# Autodesk Inventor assembly: OpenROV_Dev_EChassis
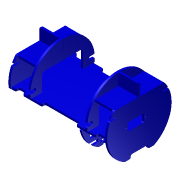
[picture p0: Inventor's stored thumbnail of the model, 180x180]
Saved by Autodesk Inventor 2012 (Build 160160000, 160)
## iProperties
Created: 2012-07-04
Part Number: OpenROV_Dev_EChassis
Document SubType Name: Assembly
Designer: user
Author: user
## Documents named in this file (9)
- C:\Users\user\Desktop\CLEAN ME\OpenROV\openrov-hardware\OpenROV 2.3.2 Dev\OpenROV_Dev_EChassis.iam
- C:\Users\user\Desktop\CLEAN ME\OpenROV\openrov-hardware\OpenROV 2.3.2 Dev\OpenROV_Dev_EChassis_Main_Plate.ipt
- C:\Users\user\Desktop\CLEAN ME\OpenROV\openrov-hardware\OpenROV 2.3.2 Dev\OpenROV_Dev_EChassis_Blinder.ipt
- C:\Users\user\Desktop\CLEAN ME\OpenROV\openrov-hardware\OpenROV 2.3.2 Dev\OpenROV_Dev_EChassis_Servo_Plate.ipt
- C:\Users\user\Desktop\CLEAN ME\OpenROV\openrov-hardware\OpenROV 2.3.2 Dev\OpenROV_Dev_EChassis_Plug_Mount.ipt
- C:\Users\user\Desktop\CLEAN ME\OpenROV\openrov-hardware\OpenROV 2.3.2 Dev\OpenROV_Dev_EChassis_Seperator.ipt
- C:\Users\user\Desktop\CLEAN ME\OpenROV\openrov-hardware\OpenROV 2.3.2 Dev\OpenROV_Dev_EChassis_Pivot_Plate.ipt
- C:\Users\user\Desktop\CLEAN ME\OpenROV\openrov-hardware\OpenROV 2.3.2 Dev\OpenROV_Dev_EChassis_Light_Plate.ipt
- C:\Users\user\Desktop\CLEAN ME\OpenROV\openrov-hardware\OpenROV 2.3.2 Dev\OpenROV_Dev_EChassis_Horz_Blinder.ipt
## Components (12 placed, 8 different names)
1. OpenROV_Dev_EChassis_Main_Plate:1 — Mate:1, Mate:2, Mate:3, Mate:4, Mate:5, Mate:6, Mate:7, Mate:8, Mate:9, Mate:10, Mate:11, Mate:12, Mate:13, Mate:14, Mate:15, Mate:16, Mate:19, Mate:20, Mate:21
2. OpenROV_Dev_EChassis_Blinder:1 — Mate:1, Mate:2, Mate:3, Mate:26, Mate:32
3. OpenROV_Dev_EChassis_Blinder:2 — Mate:4, Mate:5, Mate:6, Mate:22, Mate:29
4. OpenROV_Dev_EChassis_Servo_Plate:1 — Mate:7, Mate:8, Mate:9, Mate:23, Mate:24
5. OpenROV_Dev_EChassis_Plug_Mount:1 — Mate:10, Mate:11, Mate:12, Mate:17, Mate:18
6. OpenROV_Dev_EChassis_Seperator:1 — Mate:13, Mate:16, Mate:17
7. OpenROV_Dev_EChassis_Seperator:2 — Mate:14, Mate:15, Mate:18
8. OpenROV_Dev_EChassis_Pivot_Plate:1 — Mate:19, Mate:20, Mate:21, Mate:25, Mate:27
9. OpenROV_Dev_EChassis_Light_Plate:1 — Mate:22, Mate:23, Mate:24, Mate:28, Mate:30
10. OpenROV_Dev_EChassis_Light_Plate:2 — Mate:25, Mate:26, Mate:27, Mate:31, Mate:33
11. OpenROV_Dev_EChassis_Horz_Blinder:1 — Mate:31, Mate:32, Mate:33
12. OpenROV_Dev_EChassis_Horz_Blinder:2 — Mate:28, Mate:29, Mate:30
## Relationships (33: Mate 33)
- Mate:1: OpenROV_Dev_EChassis_Main_Plate:1 ↔ OpenROV_Dev_EChassis_Blinder:1
- Mate:2: OpenROV_Dev_EChassis_Main_Plate:1 ↔ OpenROV_Dev_EChassis_Blinder:1
- Mate:3: OpenROV_Dev_EChassis_Main_Plate:1 ↔ OpenROV_Dev_EChassis_Blinder:1
- Mate:4: OpenROV_Dev_EChassis_Main_Plate:1 ↔ OpenROV_Dev_EChassis_Blinder:2
- Mate:5: OpenROV_Dev_EChassis_Main_Plate:1 ↔ OpenROV_Dev_EChassis_Blinder:2
- Mate:6: OpenROV_Dev_EChassis_Main_Plate:1 ↔ OpenROV_Dev_EChassis_Blinder:2
- Mate:7: OpenROV_Dev_EChassis_Main_Plate:1 ↔ OpenROV_Dev_EChassis_Servo_Plate:1
- Mate:8: OpenROV_Dev_EChassis_Main_Plate:1 ↔ OpenROV_Dev_EChassis_Servo_Plate:1
- Mate:9: OpenROV_Dev_EChassis_Main_Plate:1 ↔ OpenROV_Dev_EChassis_Servo_Plate:1
- Mate:10: OpenROV_Dev_EChassis_Main_Plate:1 ↔ OpenROV_Dev_EChassis_Plug_Mount:1
- Mate:11: OpenROV_Dev_EChassis_Main_Plate:1 ↔ OpenROV_Dev_EChassis_Plug_Mount:1
- Mate:12: OpenROV_Dev_EChassis_Main_Plate:1 ↔ OpenROV_Dev_EChassis_Plug_Mount:1
- Mate:13: OpenROV_Dev_EChassis_Main_Plate:1 ↔ OpenROV_Dev_EChassis_Seperator:1
- Mate:14: OpenROV_Dev_EChassis_Main_Plate:1 ↔ OpenROV_Dev_EChassis_Seperator:2
- Mate:15: OpenROV_Dev_EChassis_Main_Plate:1 ↔ OpenROV_Dev_EChassis_Seperator:2
- Mate:16: OpenROV_Dev_EChassis_Main_Plate:1 ↔ OpenROV_Dev_EChassis_Seperator:1
- Mate:17: OpenROV_Dev_EChassis_Plug_Mount:1 ↔ OpenROV_Dev_EChassis_Seperator:1
- Mate:18: OpenROV_Dev_EChassis_Plug_Mount:1 ↔ OpenROV_Dev_EChassis_Seperator:2
- Mate:19: OpenROV_Dev_EChassis_Main_Plate:1 ↔ OpenROV_Dev_EChassis_Pivot_Plate:1
- Mate:20: OpenROV_Dev_EChassis_Main_Plate:1 ↔ OpenROV_Dev_EChassis_Pivot_Plate:1
- Mate:21: OpenROV_Dev_EChassis_Main_Plate:1 ↔ OpenROV_Dev_EChassis_Pivot_Plate:1
- Mate:22: OpenROV_Dev_EChassis_Blinder:2 ↔ OpenROV_Dev_EChassis_Light_Plate:1
- Mate:23: OpenROV_Dev_EChassis_Servo_Plate:1 ↔ OpenROV_Dev_EChassis_Light_Plate:1
- Mate:24: OpenROV_Dev_EChassis_Servo_Plate:1 ↔ OpenROV_Dev_EChassis_Light_Plate:1
- Mate:25: OpenROV_Dev_EChassis_Pivot_Plate:1 ↔ OpenROV_Dev_EChassis_Light_Plate:2
- Mate:26: OpenROV_Dev_EChassis_Blinder:1 ↔ OpenROV_Dev_EChassis_Light_Plate:2
- Mate:27: OpenROV_Dev_EChassis_Pivot_Plate:1 ↔ OpenROV_Dev_EChassis_Light_Plate:2
- Mate:28: OpenROV_Dev_EChassis_Light_Plate:1 ↔ OpenROV_Dev_EChassis_Horz_Blinder:2
- Mate:29: OpenROV_Dev_EChassis_Blinder:2 ↔ OpenROV_Dev_EChassis_Horz_Blinder:2
- Mate:30: OpenROV_Dev_EChassis_Light_Plate:1 ↔ OpenROV_Dev_EChassis_Horz_Blinder:2
- Mate:31: OpenROV_Dev_EChassis_Light_Plate:2 ↔ OpenROV_Dev_EChassis_Horz_Blinder:1
- Mate:32: OpenROV_Dev_EChassis_Blinder:1 ↔ OpenROV_Dev_EChassis_Horz_Blinder:1
- Mate:33: OpenROV_Dev_EChassis_Light_Plate:2 ↔ OpenROV_Dev_EChassis_Horz_Blinder:1
